# Autodesk Inventor assembly: Assembly2
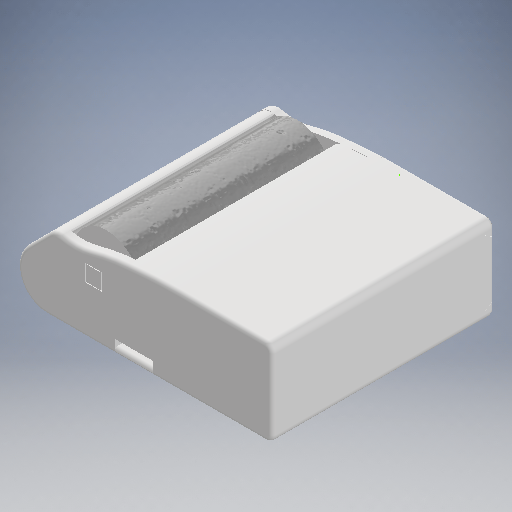
[picture p0: Inventor's stored thumbnail of the model, 512x512]
Saved by Autodesk Inventor 2025.2 (Build 292293000, 293)
## iProperties
Created: 2025-02-14
Part Number: Assembly2
Document SubType Name: Assembly
Designer: Alex
Author: Alex
## Documents named in this file (6)
- C:\Shared\alex-bartella-schoolwork\4b03\a1\Assembly2.iam
- C:\Shared\alex-bartella-schoolwork\4b03\a1\roller.ipt
- C:\Shared\alex-bartella-schoolwork\4b03\a1\tank.ipt
- C:\Shared\alex-bartella-schoolwork\4b03\a1\shaft.ipt
- C:\Shared\alex-bartella-schoolwork\4b03\a1\door.ipt
- C:\Shared\alex-bartella-schoolwork\4b03\a1\Part7.ipt
## Components (5 placed, 5 different names)
1. roller:1 — Mate:1
2. tank:1 — Mate:2, Mate:3, Flush:4, Mate:4, Flush:5, Mate:5
3. shaft:1 — Mate:1, Mate:2, Mate:3
4. door:1 — Flush:4
5. Part7:1 — Mate:4, Flush:5, Mate:5
## Relationships (7: Mate 5, Flush 2)
- Mate:1: roller:1 ↔ shaft:1
- Mate:2 (0.35 mm): tank:1 ↔ shaft:1
- Mate:3: tank:1 ↔ shaft:1
- Flush:4: tank:1 ↔ door:1
- Mate:4: tank:1 ↔ Part7:1
- Flush:5: tank:1 ↔ Part7:1
- Mate:5: tank:1 ↔ Part7:1
